# Autodesk Inventor assembly: мотор левая_MIR
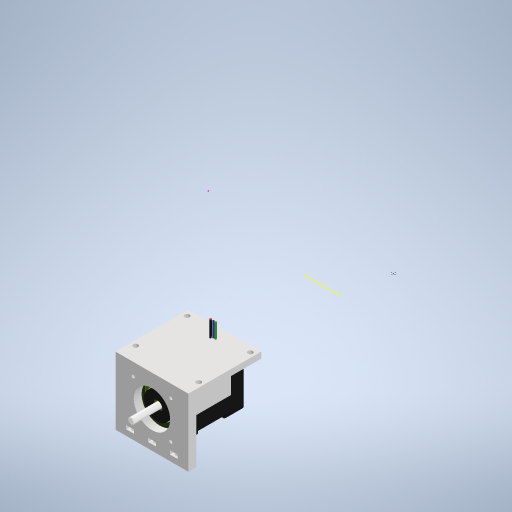
[picture p0: Inventor's stored thumbnail of the model, 512x512]
Saved by Autodesk Inventor 2024.2 (Build 282272000, 272)
## iProperties
Created: 2025-11-21
Part Number: мотор левая_MIR
Document SubType Name: Assembly
Designer: katya_notebook
Mass: 33.357 g
Surface Area: 174.781 cm^2
Volume: 33.357 cm^3
Density: 1 g/cm^3
Author: katya_notebook
## Documents named in this file (3)
- D:\alletz\construction\мотор левая_MIR.iam
- D:\alletz\construction\крепление_MIR.ipt
- D:\alletz\construction\toothed_rack\Nema 17 Stepper.ipt
## Components (2 placed, 2 different names)
1. Nema 17 Stepper:1 — С поворотом:1
2. крепление_MIR:1 — С поворотом:1
## Relationships (1: RevoluteJoint 1)
- С поворотом:1 [RevoluteJoint]: Nema 17 Stepper:1 ↔ крепление_MIR:1
